# Autodesk Inventor assembly: Mass 1
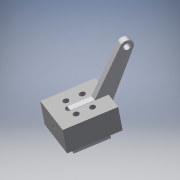
[picture p0: Inventor's stored thumbnail of the model, 180x180]
Saved by Autodesk Inventor 2016 (Build 200138000, 138)
## iProperties
Created: 2015-06-08
Part Number: Mass 1
Document SubType Name: Assembly
Designer: Dennis
Author: Dennis
## Documents named in this file (4)
- C:\Users\Dennis\Dropbox\NI Work\NI Slider Crank\Assemblies\Mass 1.iam
- C:\Users\Dennis\Dropbox\NI Work\NI Slider Crank\Parts\Carriage - 9829K300.ipt
- C:\Users\Dennis\Dropbox\NI Work\NI Slider Crank\Parts\Mass 1 Insert.ipt
- C:\Users\Dennis\Dropbox\NI Work\NI Slider Crank\Parts\Mass 1.ipt
## Components (3 placed, 3 different names)
1. Carriage - 9829K300:1 — Mate:4, Mate:5, Mate:6
2. Mass 1 Insert:1 — Mate:1, Mate:2, Mate:3
3. Mass 1:1 — Mate:1, Mate:2, Mate:3, Mate:4, Mate:5, Mate:6
## Relationships (6: Mate 6)
- Mate:1: Mass 1 Insert:1 ↔ Mass 1:1
- Mate:2: Mass 1 Insert:1 ↔ Mass 1:1
- Mate:3: Mass 1 Insert:1 ↔ Mass 1:1
- Mate:4: Carriage - 9829K300:1 ↔ Mass 1:1
- Mate:5: Carriage - 9829K300:1 ↔ Mass 1:1
- Mate:6: Carriage - 9829K300:1 ↔ Mass 1:1
